# Autodesk Inventor assembly: Assembly1
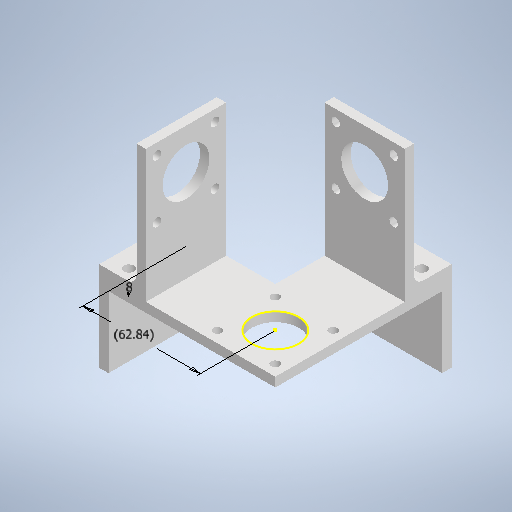
[picture p0: Inventor's stored thumbnail of the model, 512x512]
Saved by Autodesk Inventor 2025 (Build 290162010, 162A)
## iProperties
Created: 2025-02-16
Part Number: Assembly1
Document SubType Name: Assembly
Designer: aduwa
Author: aduwa
## Documents named in this file (3)
- C:\Users\aduwa\OneDrive\Documents\PROJECTS\2025\CAPSTONE\V1\Assembly1.iam
- C:\Users\aduwa\OneDrive\Documents\PROJECTS\2025\CAPSTONE\V1\test_base.ipt
- C:\Users\aduwa\OneDrive\Documents\PROJECTS\2025\CAPSTONE\V1\motor_holder.ipt
## Components (3 placed, 2 different names)
1. test_base:1 — Mate:1, Mate:2, Mate:3, Mate:4, Mate:5, Mate:6
2. motor_holder:1 — Mate:1, Mate:2, Mate:3
3. motor_holder:2 — Mate:4, Mate:5, Mate:6
## Relationships (6: Mate 6)
- Mate:1: test_base:1 ↔ motor_holder:1
- Mate:2: test_base:1 ↔ motor_holder:1
- Mate:3: test_base:1 ↔ motor_holder:1
- Mate:4: test_base:1 ↔ motor_holder:2
- Mate:5: test_base:1 ↔ motor_holder:2
- Mate:6: test_base:1 ↔ motor_holder:2
